# Autodesk Inventor assembly: Hafele Handle 115.70
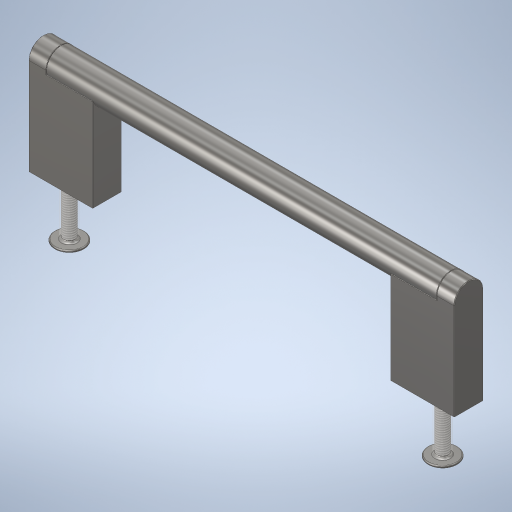
[picture p0: Inventor's stored thumbnail of the model, 512x512]
Saved by Autodesk Inventor 2024 (Build 280153000, 153)
## iProperties
RuleStatus: InUse
Created: 2023-02-13
Part Number: Hafele Handle 115.70
Document SubType Name: Assembly
Designer: sauliusd
Author: sauliusd
## Documents named in this file (4)
- C:\W4INV 2024 Design\SMART HARDWARE\Handles\Hafele Handle 115.70\Parts\Hafele Handle 115.70.iam
- C:\W4INV 2024 Design\PROJECTS\MODEL STATE LIBRARY COMPONENTS\Handles\Hafele Handle 115.70.ipt
- C:\W4INV 2024 Design\LIBRARY\Handles\M4 Threated Screw.ipt
- C:\W4INV 2024 Design\SMART HARDWARE\Handles\Hafele Handle 115.70\Parts\Hafele Handle 115.70 Hole.ipt
## Components (5 placed, 4 different names)
1. Hafele Handle — Insert:1, Insert:2, Flush:1, Flush:2, Mate:1
2. Hole — Insert:1, Insert:3
3. Hafele Handle 115.70 Hole:2 — Insert:2, Insert:4
4. M4 Threated Screw:1 — Insert:3
5. M4 Threated Screw:2 — Insert:4
## Relationships (7: Insert 4, Flush 2, Mate 1)
- Insert:1: Hafele Handle ↔ Hole
- Insert:2: Hafele Handle ↔ Hafele Handle 115.70 Hole:2
- Insert:3: Hole ↔ M4 Threated Screw:1
- Insert:4: Hafele Handle 115.70 Hole:2 ↔ M4 Threated Screw:2
- Flush:1: Hafele Handle
- Flush:2: Hafele Handle
- Mate:1: Hafele Handle
## Named parameters: NestledBoardT = 18 mm
